# Autodesk Inventor assembly: Prensa_Hidraulica
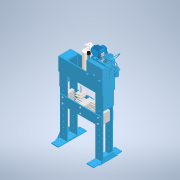
[picture p0: Inventor's stored thumbnail of the model, 180x180]
Saved by Autodesk Inventor 2021 (Build 250183000, 183)
## iProperties
Created: 2020-01-15
Part Number: Prensa_Hidraulica
Document SubType Name: Assembly
Designer: Nelson
Sending System: SolidWorks 2020
Last Author: Micro
Last Saved: 2020-01-16
Author: Nelson
## Documents named in this file (11)
- D:\Nelson\Documentos\Inventor\PrensaHidraulica_Automatizada\Prensa_Hidraulica.iam
- Prensa_Hidraulica.iam
- D:\Nelson\Documentos\Inventor\PrensaHidraulica_Automatizada\Estructura.iam
- D:\Nelson\Documentos\Inventor\PrensaHidraulica_Automatizada\Cilindro neumatico.ipt
- D:\Nelson\Documentos\Inventor\PrensaHidraulica_Automatizada\Bomba Hidraulica.ipt
- D:\Nelson\Documentos\Inventor\PrensaHidraulica_Automatizada\Soporte barras.ipt
- D:\Nelson\Documentos\Inventor\PrensaHidraulica_Automatizada\Barra de deslizamiento.ipt
- D:\Nelson\Documentos\Inventor\PrensaHidraulica_Automatizada\Ensamble Mecanismo cilindro.iam
- D:\Nelson\Documentos\Inventor\PrensaHidraulica_Automatizada\1808236 DFPI-100-280-ND2P-E-P-G2---(0).iam
- D:\Nelson\Documentos\Inventor\PrensaHidraulica_Automatizada\Soporte mesa.ipt
- D:\Nelson\Documentos\Inventor\PrensaHidraulica_Automatizada\PH 013.ipt
## Components (17 placed, 9 different names)
1. Cilindro neumatico:1 — Mate:2, Mate:3
2. Bomba Hidraulica:1 — Mate:1, Flush:1, Flush:2
3. Soporte barras:1 — Mate:4, Mate:19, Mate:22, Mate:24
4. Soporte barras:2 — Mate:5, Mate:20, Mate:21, Flush:3, Mate:23, Flush:4
5. Barra de deslizamiento:1 — Mate:21, Mate:22, Flush:3, Mate:26, Mate:28
6. Barra de deslizamiento:2 — Mate:23, Mate:24, Flush:4, Mate:25, Mate:27
7. Ensamble mecanismo cilindro:1 [sub-assembly] — Mate:25, Mate:26
8. Ensamble mecanismo cilindro:2 [sub-assembly] — Mate:27, Mate:28
9. 1808236 DFPI-100-280-ND2P-E-P-G2---(0):1 [sub-assembly]
10. Soporte mesa:1 — Mate:29, Mate:30, Mate:31
11. PH 013:1 — Mate:36, Mate:37
12. PH 013:2 — Mate:38, Mate:39
13. PH 013:3 — Mate:40, Mate:42
14. PH 013:4 — Mate:41, Mate:43
15. PH 013:5 — Mate:34, Mate:35
16. PH 013:6 — Mate:32, Mate:33
17. Estructura:1 [sub-assembly] — Mate:1, Flush:1, Flush:2, Mate:2, Mate:3, Mate:4, Mate:5, Mate:19, Mate:20, Mate:29, Mate:30, Mate:31, Mate:32, Mate:33, Mate:34, Mate:35, Mate:36, Mate:37, Mate:38, Mate:39, Mate:40, Mate:41, Mate:42, Mate:43
## Relationships (34: Mate 30, Flush 4)
- Mate:1: Bomba Hidraulica:1 ↔ Estructura:1
- Flush:1: Bomba Hidraulica:1 ↔ Estructura:1
- Flush:2: Bomba Hidraulica:1 ↔ Estructura:1
- Mate:2: Cilindro neumatico:1 ↔ Estructura:1
- Mate:3: Cilindro neumatico:1 ↔ Estructura:1
- Mate:4: Soporte barras:1 ↔ Estructura:1
- Mate:5: Soporte barras:2 ↔ Estructura:1
- Mate:19: Soporte barras:1 ↔ Estructura:1
- Mate:20: Soporte barras:2 ↔ Estructura:1
- Mate:21: Soporte barras:2 ↔ Barra de deslizamiento:1
- Mate:22: Soporte barras:1 ↔ Barra de deslizamiento:1
- Flush:3: Soporte barras:2 ↔ Barra de deslizamiento:1
- Mate:23: Soporte barras:2 ↔ Barra de deslizamiento:2
- Mate:24: Soporte barras:1 ↔ Barra de deslizamiento:2
- Flush:4: Soporte barras:2 ↔ Barra de deslizamiento:2
- Mate:25: Barra de deslizamiento:2 ↔ Ensamble mecanismo cilindro:1
- Mate:26: Barra de deslizamiento:1 ↔ Ensamble mecanismo cilindro:1
- Mate:27: Barra de deslizamiento:2 ↔ Ensamble mecanismo cilindro:2
- Mate:28: Barra de deslizamiento:1 ↔ Ensamble mecanismo cilindro:2
- Mate:29: Soporte mesa:1 ↔ Estructura:1
- Mate:30: Soporte mesa:1 ↔ Estructura:1
- Mate:31: Soporte mesa:1 ↔ Estructura:1
- Mate:32: PH 013:6 ↔ Estructura:1
- Mate:33: PH 013:6 ↔ Estructura:1
- Mate:34: PH 013:5 ↔ Estructura:1
- Mate:35: PH 013:5 ↔ Estructura:1
- Mate:36: PH 013:1 ↔ Estructura:1
- Mate:37: PH 013:1 ↔ Estructura:1
- Mate:38: PH 013:2 ↔ Estructura:1
- Mate:39: PH 013:2 ↔ Estructura:1
- Mate:40: PH 013:3 ↔ Estructura:1
- Mate:41: PH 013:4 ↔ Estructura:1
- Mate:42: PH 013:3 ↔ Estructura:1
- Mate:43: PH 013:4 ↔ Estructura:1
